# Autodesk Inventor assembly: GE-20100
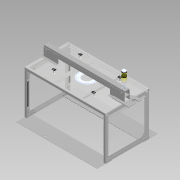
[picture p0: Inventor's stored thumbnail of the model, 180x180]
Saved by Autodesk Inventor 2020.1 (Build 241239000, 239)
## iProperties
Created: 2019-10-14
Part Number: GE-20100
Document SubType Name: Assembly
Designer: Phillips Lenovo
Author: Phillips Lenovo
Revision Number: ANY
## Documents named in this file (33)
- D:\FIRST 2020\FRC 2020\FRC Field 2020\Parts\GE-20100.iam
- D:\FIRST 2020\FRC 2020\FRC Field 2020\Parts\GE-20102.iam
- D:\FIRST 2020\FRC 2020\FRC Field 2020\Parts\GE-20101.iam
- D:\FIRST 2020\FRC 2020\FRC Field 2020\Parts\GE-20101_1.iam
- D:\FIRST 2020\FRC 2020\FRC Field 2020\Parts\GE-20114.ipt
- D:\FIRST 2020\FRC 2020\FRC Field 2020\Parts\GE-20115.ipt
- D:\FIRST 2020\FRC 2020\FRC Field 2020\Parts\am-0516 0.375'''' id bearing, shielded (R6ZZ).step.ipt
- D:\FIRST 2020\FRC 2020\FRC Field 2020\Parts\GE-20121.ipt
- D:\FIRST 2020\FRC 2020\FRC Field 2020\Parts\91255A617_ALLOY STEEL BUTTON-HEAD SOCKET CAP SCREW_91255A617.ipt
- D:\FIRST 2020\FRC 2020\FRC Field 2020\Parts\92511A109_ALUM UNTHRD SPACER_92511A109.ipt
- D:\FIRST 2020\FRC 2020\FRC Field 2020\Parts\855t-bpm10.ipt
- D:\FIRST 2020\FRC 2020\FRC Field 2020\Parts\91253A540_ALLOY STEEL FLAT-HEAD SOCKET CAP SCREW_91253A540.ipt
- D:\FIRST 2020\FRC 2020\FRC Field 2020\Parts\92949A267_18-8 SS BUTTON HEAD HEX DRIVE SCREW_92949A267.ipt
- D:\FIRST 2020\FRC 2020\FRC Field 2020\Parts\91253A550_ALLOY STEEL FLAT-HEAD SOCKET CAP SCREW_91253A550.ipt
- D:\FIRST 2020\FRC 2020\FRC Field 2020\Parts\GE-20140_hinged top.iam
- D:\FIRST 2020\FRC 2020\FRC Field 2020\Parts\90985A126_HIGH PROFILE PUSH-BUTTON QUICK-RELEASE PIN_90985A126.ipt
- D:\FIRST 2020\FRC 2020\FRC Field 2020\Parts\GE-20123.ipt
- D:\FIRST 2020\FRC 2020\FRC Field 2020\Parts\GE-20141.ipt
- D:\FIRST 2020\FRC 2020\FRC Field 2020\Parts\46CLR.stp.ipt
- D:\FIRST 2020\FRC 2020\FRC Field 2020\Parts\GE-20142.ipt
- D:\FIRST 2020\FRC 2020\FRC Field 2020\Parts\GE-20143.ipt
- D:\FIRST 2020\FRC 2020\FRC Field 2020\Parts\90272A835_ZINC-PLTD STL PAN HEAD PHILLIPS MACHINE SCREW_90272A835.ipt
- D:\FIRST 2020\FRC 2020\FRC Field 2020\Parts\90631A411_LOW-STRENGTH STEEL NYLON-INSERT LOCKNUT_90631A411.ipt
- D:\FIRST 2020\FRC 2020\FRC Field 2020\Parts\GE-20150.iam
- D:\FIRST 2020\FRC 2020\FRC Field 2020\Parts\95615A120_ZINC-PLATED GRADE 5 STL NYLON-INSERT LOCKNUT_95615A120.ipt
- D:\FIRST 2020\FRC 2020\FRC Field 2020\Parts\95615A140_ZINC-PLATED GRADE 5 STL NYLON-INSERT LOCKNUT_95615A140.ipt
- D:\FIRST 2020\FRC 2020\FRC Field 2020\Parts\Hook_1_15.ipt
- D:\FIRST 2020\FRC 2020\FRC Field 2020\Parts\Loop_1_15.ipt
- D:\FIRST 2020\FRC 2020\FRC Field 2020\Parts\Hook_4_55.ipt
- D:\FIRST 2020\FRC 2020\FRC Field 2020\Parts\855t_module.iam
- D:\FIRST 2020\FRC 2020\FRC Field 2020\Parts\855t_module_1.iam
- D:\FIRST 2020\FRC 2020\FRC Field 2020\Parts\855T-CAP.ipt
- 46CLR.stp
## Components (139 placed, 139 different names)
1. GE-20102_2610 [sub-assembly]
2. GE-20101_2611 [sub-assembly]
3. GE-20101_2612 [sub-assembly]
4. GE-20114_2613 — Flush:1, Flush:2
5. GE-20115_2615
6. GE-20115_2616
7. GE-20121_2625
8. GE-20121_2626
9. GE-20121_2627
10. GE-20121_2628
11. 855t-bpm10_2636
12. GE-20140_hinged top_2653 [sub-assembly]
13. GE-20123_2655
14. GE-20123_2656
15. GE-20141_2657
16. GE-20141_2658
17. 46CLR.stp_2659
18. GE-20142_2660
19. GE-20143_2677
20. GE-20150_2722 [sub-assembly]
21. 855t_module_2751 [sub-assembly]
22. 855t_module_2752 [sub-assembly]
23. 855T-CAP_2753
24. Hook_1_15_2739
25. Hook_1_15_2740
26. Hook_1_15_2741
27. Hook_1_15_2742
28. Loop_1_15_2743
29. Loop_1_15_2744
30. Loop_1_15_2745
31. Loop_1_15_2746
32. Hook_4_55_2747
33. Hook_4_55_2748
34. Hook_4_55_2749
35. Hook_4_55_2750
36. 95615A120_ZINC-PLATED GRADE 5 STL NYLON-INSERT LOCKNUT_95615A120_2730
37. am-0516 0.375'''' id bearing, shielded (R6ZZ).step_2617
38. am-0516 0.375'''' id bearing, shielded (R6ZZ).step_2618
39. am-0516 0.375'''' id bearing, shielded (R6ZZ).step_2619
40. am-0516 0.375'''' id bearing, shielded (R6ZZ).step_2620
41. am-0516 0.375'''' id bearing, shielded (R6ZZ).step_2621
42. am-0516 0.375'''' id bearing, shielded (R6ZZ).step_2622
43. am-0516 0.375'''' id bearing, shielded (R6ZZ).step_2623
44. am-0516 0.375'''' id bearing, shielded (R6ZZ).step_2624
45. 90985A126_HIGH PROFILE PUSH-BUTTON QUICK-RELEASE PIN_90985A126_2654
46. 91255A617_ALLOY STEEL BUTTON-HEAD SOCKET CAP SCREW_91255A617_2629
47. 92511A109_ALUM UNTHRD SPACER_92511A109_2630
48. 92511A109_ALUM UNTHRD SPACER_92511A109_2631
49. 92511A109_ALUM UNTHRD SPACER_92511A109_2632
50. 91255A617_ALLOY STEEL BUTTON-HEAD SOCKET CAP SCREW_91255A617_2633
51. 91255A617_ALLOY STEEL BUTTON-HEAD SOCKET CAP SCREW_91255A617_2634
52. 91255A617_ALLOY STEEL BUTTON-HEAD SOCKET CAP SCREW_91255A617_2635
53. 91253A540_ALLOY STEEL FLAT-HEAD SOCKET CAP SCREW_91253A540_2637
54. 91253A540_ALLOY STEEL FLAT-HEAD SOCKET CAP SCREW_91253A540_2638
55. 91253A540_ALLOY STEEL FLAT-HEAD SOCKET CAP SCREW_91253A540_2639
56. 91253A540_ALLOY STEEL FLAT-HEAD SOCKET CAP SCREW_91253A540_2640
57. 91253A540_ALLOY STEEL FLAT-HEAD SOCKET CAP SCREW_91253A540_2641
58. 91253A540_ALLOY STEEL FLAT-HEAD SOCKET CAP SCREW_91253A540_2642
59. 91253A540_ALLOY STEEL FLAT-HEAD SOCKET CAP SCREW_91253A540_2643
60. 91253A540_ALLOY STEEL FLAT-HEAD SOCKET CAP SCREW_91253A540_2644
61. 92949A267_18-8 SS BUTTON HEAD HEX DRIVE SCREW_92949A267_2645
62. 92949A267_18-8 SS BUTTON HEAD HEX DRIVE SCREW_92949A267_2646
63. 92949A267_18-8 SS BUTTON HEAD HEX DRIVE SCREW_92949A267_2647
64. 92949A267_18-8 SS BUTTON HEAD HEX DRIVE SCREW_92949A267_2648
65. 91253A550_ALLOY STEEL FLAT-HEAD SOCKET CAP SCREW_91253A550_2649
66. 91253A550_ALLOY STEEL FLAT-HEAD SOCKET CAP SCREW_91253A550_2650
67. 91253A550_ALLOY STEEL FLAT-HEAD SOCKET CAP SCREW_91253A550_2651
68. 91253A550_ALLOY STEEL FLAT-HEAD SOCKET CAP SCREW_91253A550_2652
69. 90985A126_HIGH PROFILE PUSH-BUTTON QUICK-RELEASE PIN_90985A126_2661
70. 90985A126_HIGH PROFILE PUSH-BUTTON QUICK-RELEASE PIN_90985A126_2662
71. 90985A126_HIGH PROFILE PUSH-BUTTON QUICK-RELEASE PIN_90985A126_2663
72. 92949A267_18-8 SS BUTTON HEAD HEX DRIVE SCREW_92949A267_2664
73. 92949A267_18-8 SS BUTTON HEAD HEX DRIVE SCREW_92949A267_2665
74. 92949A267_18-8 SS BUTTON HEAD HEX DRIVE SCREW_92949A267_2666
75. 92949A267_18-8 SS BUTTON HEAD HEX DRIVE SCREW_92949A267_2667
76. 92949A267_18-8 SS BUTTON HEAD HEX DRIVE SCREW_92949A267_2668
77. 92949A267_18-8 SS BUTTON HEAD HEX DRIVE SCREW_92949A267_2669
78. 92949A267_18-8 SS BUTTON HEAD HEX DRIVE SCREW_92949A267_2670
79. 92949A267_18-8 SS BUTTON HEAD HEX DRIVE SCREW_92949A267_2671
80. 92511A109_ALUM UNTHRD SPACER_92511A109_2676
81. 90272A835_ZINC-PLTD STL PAN HEAD PHILLIPS MACHINE SCREW_90272A835_2678
82. 90272A835_ZINC-PLTD STL PAN HEAD PHILLIPS MACHINE SCREW_90272A835_2679
83. 90272A835_ZINC-PLTD STL PAN HEAD PHILLIPS MACHINE SCREW_90272A835_2680
84. 90272A835_ZINC-PLTD STL PAN HEAD PHILLIPS MACHINE SCREW_90272A835_2681
85. 90631A411_LOW-STRENGTH STEEL NYLON-INSERT LOCKNUT_90631A411_2682
86. 90631A411_LOW-STRENGTH STEEL NYLON-INSERT LOCKNUT_90631A411_2683
87. 90631A411_LOW-STRENGTH STEEL NYLON-INSERT LOCKNUT_90631A411_2684
88. 90631A411_LOW-STRENGTH STEEL NYLON-INSERT LOCKNUT_90631A411_2685
89. 90631A411_LOW-STRENGTH STEEL NYLON-INSERT LOCKNUT_90631A411_2686
90. 90631A411_LOW-STRENGTH STEEL NYLON-INSERT LOCKNUT_90631A411_2687
91. 90631A411_LOW-STRENGTH STEEL NYLON-INSERT LOCKNUT_90631A411_2688
92. 90631A411_LOW-STRENGTH STEEL NYLON-INSERT LOCKNUT_90631A411_2689
93. 90631A411_LOW-STRENGTH STEEL NYLON-INSERT LOCKNUT_90631A411_2690
94. 90631A411_LOW-STRENGTH STEEL NYLON-INSERT LOCKNUT_90631A411_2691
95. 90631A411_LOW-STRENGTH STEEL NYLON-INSERT LOCKNUT_90631A411_2692
96. 90631A411_LOW-STRENGTH STEEL NYLON-INSERT LOCKNUT_90631A411_2693
97. 90631A411_LOW-STRENGTH STEEL NYLON-INSERT LOCKNUT_90631A411_2694
98. 90631A411_LOW-STRENGTH STEEL NYLON-INSERT LOCKNUT_90631A411_2695
99. 90631A411_LOW-STRENGTH STEEL NYLON-INSERT LOCKNUT_90631A411_2696
100. 90631A411_LOW-STRENGTH STEEL NYLON-INSERT LOCKNUT_90631A411_2697
101. 90631A411_LOW-STRENGTH STEEL NYLON-INSERT LOCKNUT_90631A411_2698
102. 90631A411_LOW-STRENGTH STEEL NYLON-INSERT LOCKNUT_90631A411_2699
103. 90631A411_LOW-STRENGTH STEEL NYLON-INSERT LOCKNUT_90631A411_2700
104. 90631A411_LOW-STRENGTH STEEL NYLON-INSERT LOCKNUT_90631A411_2701
105. 92949A267_18-8 SS BUTTON HEAD HEX DRIVE SCREW_92949A267_2702
106. 92949A267_18-8 SS BUTTON HEAD HEX DRIVE SCREW_92949A267_2703
107. 92949A267_18-8 SS BUTTON HEAD HEX DRIVE SCREW_92949A267_2704
108. 92949A267_18-8 SS BUTTON HEAD HEX DRIVE SCREW_92949A267_2705
109. 92949A267_18-8 SS BUTTON HEAD HEX DRIVE SCREW_92949A267_2706
110. 92949A267_18-8 SS BUTTON HEAD HEX DRIVE SCREW_92949A267_2707
111. 92949A267_18-8 SS BUTTON HEAD HEX DRIVE SCREW_92949A267_2708
112. 92949A267_18-8 SS BUTTON HEAD HEX DRIVE SCREW_92949A267_2709
113. 92949A267_18-8 SS BUTTON HEAD HEX DRIVE SCREW_92949A267_2710
114. 92949A267_18-8 SS BUTTON HEAD HEX DRIVE SCREW_92949A267_2711
115. 92949A267_18-8 SS BUTTON HEAD HEX DRIVE SCREW_92949A267_2712
116. 92949A267_18-8 SS BUTTON HEAD HEX DRIVE SCREW_92949A267_2713
117. 90631A411_LOW-STRENGTH STEEL NYLON-INSERT LOCKNUT_90631A411_2714
118. 90631A411_LOW-STRENGTH STEEL NYLON-INSERT LOCKNUT_90631A411_2715
119. 90631A411_LOW-STRENGTH STEEL NYLON-INSERT LOCKNUT_90631A411_2716
120. 90631A411_LOW-STRENGTH STEEL NYLON-INSERT LOCKNUT_90631A411_2717
121. 90631A411_LOW-STRENGTH STEEL NYLON-INSERT LOCKNUT_90631A411_2718
122. 90631A411_LOW-STRENGTH STEEL NYLON-INSERT LOCKNUT_90631A411_2719
123. 90631A411_LOW-STRENGTH STEEL NYLON-INSERT LOCKNUT_90631A411_2720
124. 90631A411_LOW-STRENGTH STEEL NYLON-INSERT LOCKNUT_90631A411_2721
125. 95615A120_ZINC-PLATED GRADE 5 STL NYLON-INSERT LOCKNUT_95615A120_2723
126. 95615A120_ZINC-PLATED GRADE 5 STL NYLON-INSERT LOCKNUT_95615A120_2724
127. 95615A120_ZINC-PLATED GRADE 5 STL NYLON-INSERT LOCKNUT_95615A120_2725
128. 95615A120_ZINC-PLATED GRADE 5 STL NYLON-INSERT LOCKNUT_95615A120_2726
129. 95615A120_ZINC-PLATED GRADE 5 STL NYLON-INSERT LOCKNUT_95615A120_2727
130. 95615A120_ZINC-PLATED GRADE 5 STL NYLON-INSERT LOCKNUT_95615A120_2728
131. 95615A120_ZINC-PLATED GRADE 5 STL NYLON-INSERT LOCKNUT_95615A120_2729
132. 95615A120_ZINC-PLATED GRADE 5 STL NYLON-INSERT LOCKNUT_95615A120_2731
133. 95615A120_ZINC-PLATED GRADE 5 STL NYLON-INSERT LOCKNUT_95615A120_2732
134. 95615A120_ZINC-PLATED GRADE 5 STL NYLON-INSERT LOCKNUT_95615A120_2733
135. 95615A120_ZINC-PLATED GRADE 5 STL NYLON-INSERT LOCKNUT_95615A120_2734
136. 95615A140_ZINC-PLATED GRADE 5 STL NYLON-INSERT LOCKNUT_95615A140_2735
137. 95615A140_ZINC-PLATED GRADE 5 STL NYLON-INSERT LOCKNUT_95615A140_2736
138. 95615A140_ZINC-PLATED GRADE 5 STL NYLON-INSERT LOCKNUT_95615A140_2737
139. 95615A140_ZINC-PLATED GRADE 5 STL NYLON-INSERT LOCKNUT_95615A140_2738
## Relationships (2: Flush 2)
- Flush:1 (-381 mm): GE-20114_2613
- Flush:2 (-704.85 mm): GE-20114_2613
